# Autodesk Inventor assembly: Stewart-Base-KST-DS215
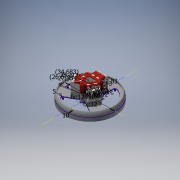
[picture p0: Inventor's stored thumbnail of the model, 180x180]
Saved by Autodesk Inventor 2018.2 (Build 222227000, 227)
## iProperties
Created: 2018-02-24
Part Number: Stewart-Base-KST-DS215
Material: Generisch
Document SubType Name: Assembly
Designer: JochenAlt
Author: JochenAlt
## Documents named in this file (5)
- D:\Projects\Donna\CAD\Stewart-Base.iam
- D:\Projects\Donna\CAD\Servo-KST-DS215MG.ipt
- D:\Projects\Donna\CAD\Messung.ipt
- D:\Projects\Donna\CAD\Servo-Arm-Head-20mm-Ball-Joint.iam
- D:\Projects\Donna\CAD\Stewart-Platform-Base2.ipt
## Components (9 placed, 4 different names)
1. Servo-KST-DS215MG:1
2. Servo-KST-DS215MG:2
3. Servo-KST-DS215MG:3
4. Servo-KST-DS215MG:4
5. Servo-KST-DS215MG:5
6. Servo-KST-DS215MG:6 — Passend:67, Passend:68
7. Servo-Arm-Head-20mm-Ball-Joint:1 [sub-assembly] — Passend:67, Passend:68
8. Messung:1 — Fluchtend:1
9. Stewart-Platform-Base2:1
## Relationships (3: Mate 2, Flush 1)
- Fluchtend:1 [Flush]: Messung:1
- Passend:67 [Mate]: Servo-KST-DS215MG:6 ↔ Servo-Arm-Head-20mm-Ball-Joint:1
- Passend:68 [Mate]: Servo-KST-DS215MG:6 ↔ Servo-Arm-Head-20mm-Ball-Joint:1
